# Autodesk Inventor assembly: differential gearbox
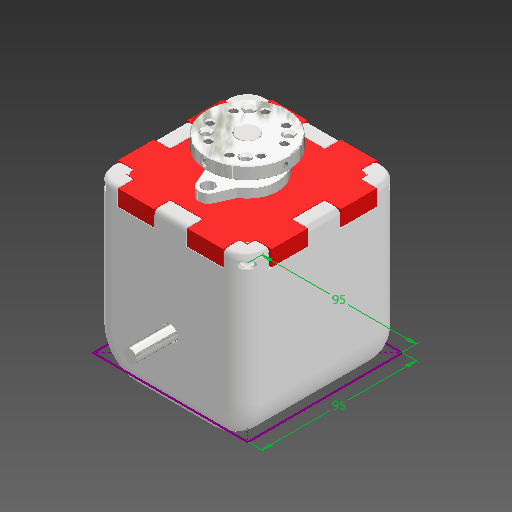
[picture p0: Inventor's stored thumbnail of the model, 512x512]
Saved by Autodesk Inventor 2020 (Build 240168000, 168)
## iProperties
Created: 2020-05-19
Part Number: differential gearbox
Document SubType Name: Assembly
Designer: stefa
Author: stefa
## Documents named in this file (10)
- D:\github_gedeeld\BeerMinder\3D-model\axis5_6\differential gearbox.iam
- D:\github_gedeeld\BeerMinder\3D-model\axis5_6\3 dubbele lagerblok en huis.ipt
- D:\github_gedeeld\BeerMinder\3D-model\axis5_6\deksel lagerblok huis.ipt
- D:\github_gedeeld\BeerMinder\3D-model\bearings\Ball Bearing 608ZZ.ipt
- D:\github_gedeeld\BeerMinder\3D-model\bearings\bloklager.ipt
- D:\github_gedeeld\BeerMinder\3D-model\axis5_6\axis5_6\Design Accelerator\Bevel Gears1.iam
- D:\github_gedeeld\BeerMinder\3D-model\axis5_6\as bevelgear.ipt
- D:\github_gedeeld\BeerMinder\3D-model\axis5_6\as naar endeffector.ipt
- D:\github_gedeeld\BeerMinder\3D-model\axis5_6\endeffector mount part.ipt
- D:\github_gedeeld\BeerMinder\3D-model\bearings\Bevel Gear11 met stelring.ipt
## Components (14 placed, 9 different names)
1. 3 dubbele lagerblok en huis:1 — Mate:1, Mate:2, Mate:3, Mate:4, Flush:1, Mate:5, Flush:2, Mate:6, Flush:3, Mate:7, Flush:4, Mate:8, Flush:5, Mate:9, Mate:10, Mate:11
2. deksel lagerblok huis:1 — Mate:9, Mate:10, Mate:11, Mate:12, Mate:13, Mate:14
3. Ball Bearing 608ZZ:1 — Mate:8, Flush:5, Mate:17
4. Ball Bearing 608ZZ:2 — Mate:4, Flush:1, Mate:18
5. Ball Bearing 608ZZ:3 — Mate:5, Flush:2, Flush:8
6. Ball Bearing 608ZZ:4 — Mate:6, Flush:3, Flush:6
7. Ball Bearing 608ZZ:5 — Mate:7, Flush:4, Flush:7
8. bloklager:1 — Mate:12, Mate:13, Mate:14, Mate:19
9. Bevel Gears:1 [sub-assembly] — Mate:15, Mate:16, Mate:20, Mate:21
10. klein tandwiel met stelring:1 — Mate:15, Mate:16
11. as bevelgear:1 — Mate:17, Flush:6, Mate:20
12. as bevelgear:2 — Mate:18, Flush:7
13. as naar endeffector:1 — Mate:19, Flush:8, Mate:21, Mate:22, Flush:9, Angle:1
14. endeffector mount part:1 — Mate:22, Flush:9, Angle:1
## Relationships (32: Mate 22, Flush 9, Angle 1)
- Mate:1: 3 dubbele lagerblok en huis:1
- Mate:2: 3 dubbele lagerblok en huis:1
- Mate:3: 3 dubbele lagerblok en huis:1
- Mate:4: 3 dubbele lagerblok en huis:1 ↔ Ball Bearing 608ZZ:2
- Flush:1: 3 dubbele lagerblok en huis:1 ↔ Ball Bearing 608ZZ:2
- Mate:5: 3 dubbele lagerblok en huis:1 ↔ Ball Bearing 608ZZ:3
- Flush:2: 3 dubbele lagerblok en huis:1 ↔ Ball Bearing 608ZZ:3
- Mate:6: 3 dubbele lagerblok en huis:1 ↔ Ball Bearing 608ZZ:4
- Flush:3: 3 dubbele lagerblok en huis:1 ↔ Ball Bearing 608ZZ:4
- Mate:7: 3 dubbele lagerblok en huis:1 ↔ Ball Bearing 608ZZ:5
- Flush:4: 3 dubbele lagerblok en huis:1 ↔ Ball Bearing 608ZZ:5
- Mate:8: 3 dubbele lagerblok en huis:1 ↔ Ball Bearing 608ZZ:1
- Flush:5: 3 dubbele lagerblok en huis:1 ↔ Ball Bearing 608ZZ:1
- Mate:9: 3 dubbele lagerblok en huis:1 ↔ deksel lagerblok huis:1
- Mate:10: 3 dubbele lagerblok en huis:1 ↔ deksel lagerblok huis:1
- Mate:11: 3 dubbele lagerblok en huis:1 ↔ deksel lagerblok huis:1
- Mate:12: deksel lagerblok huis:1 ↔ bloklager:1
- Mate:13: deksel lagerblok huis:1 ↔ bloklager:1
- Mate:14: deksel lagerblok huis:1 ↔ bloklager:1
- Mate:15: Bevel Gears:1 ↔ klein tandwiel met stelring:1
- Mate:16 (55.182 mm): Bevel Gears:1 ↔ klein tandwiel met stelring:1
- Mate:17: Ball Bearing 608ZZ:1 ↔ as bevelgear:1
- Mate:18: Ball Bearing 608ZZ:2 ↔ as bevelgear:2
- Flush:6 (-1 mm): Ball Bearing 608ZZ:4 ↔ as bevelgear:1
- Flush:7 (-1 mm): Ball Bearing 608ZZ:5 ↔ as bevelgear:2
- Mate:19: bloklager:1 ↔ as naar endeffector:1
- Flush:8 (-1 mm): Ball Bearing 608ZZ:3 ↔ as naar endeffector:1
- Mate:20: Bevel Gears:1 ↔ as bevelgear:1
- Mate:21: Bevel Gears:1 ↔ as naar endeffector:1
- Mate:22: as naar endeffector:1 ↔ endeffector mount part:1
- Flush:9: as naar endeffector:1 ↔ endeffector mount part:1
- Angle:1 (0 deg): as naar endeffector:1 ↔ endeffector mount part:1
